# Autodesk Inventor assembly: J005189
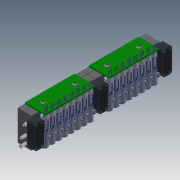
[picture p0: Inventor's stored thumbnail of the model, 180x180]
Saved by Autodesk Inventor 2020 (Build 240168000, 168)
## iProperties
RuleStatus: InUse
Created: 2015-04-18
Vendor: HHMI: JRC - ID&F
Document SubType Name: Assembly
Designer: JORDANJ
Part Number: J005189
Description: COMPONENT OF AN AUTOMATED LIQUID HANDLING MACHINE SPECIFICALLY DESIGNED FOR THE IN SITU RNA HYBRIDIZATION OF DROSOPHILA EMBRYOS
Project: P-171601
AfterDocSave0: file://Part Number Cleaner
DESIGN DEPARTMENT: HHMI: JRC - ID&F
LAB/DEPT: STERN (LAB)
REQUESTING SCIENTIST: STERN, DAVID
SPECIAL FINISH: NONE
SURFACE ROUGHNESS: N/A
ALTERED ITEM PART NUMBER: N/A
ALTERED ITEM VENDOR: N/A
ALTERED ITEM DESCRIPTION: N/A
Revision Number: 0
## Documents named in this file (4)
- C:\_WORKSPACE\DATA\PROJECTS\_PROJECTS BY LAB\STERN (LAB)\HYBRIDIZER\MCAD\MICROPLATE\24W CHEMICAL MANIFOLD ASSY.iam
- C:\_WORKSPACE\DATA\PROJECTS\_PROJECTS BY LAB\STERN (LAB)\HYBRIDIZER\MCAD\MICROPLATE\24W CHEMICAL MANIFOLD.iam
- C:\_WORKSPACE\DATA\PROJECTS\_PROJECTS BY LAB\STERN (LAB)\HYBRIDIZER\MCAD\MICROPLATE\24W CHEM MANIFOLD MOUNT.ipt
- C:\_WORKSPACE\DATA\PROJECTS\_PROJECTS BY LAB\STERN (LAB)\HYBRIDIZER\MCAD\MICROPLATE\24W CHEM MANIFOLD ORING.ipt
## Components (8 placed, 3 different names)
1. 24W CHEM MANIFOLD MOUNT:1 — Flush:6, Flush:7, Flush:8, Insert:3, Insert:4
2. 24W CHEMICAL MANIFOLD:1 [sub-assembly] — Mate:1, Flush:3, Flush:4, Flush:5, Insert:3, Insert:4, Mate:2, Mate:3, Mate:4, Flush:9, Flush:10, Flush:11
3. 24W CHEMICAL MANIFOLD:2 [sub-assembly] — Mate:1, Insert:1, Insert:2, Insert:5, Insert:6
4. 24W CHEM MANIFOLD MOUNT:2 — Insert:5, Insert:6
5. 24W CHEM MANIFOLD MOUNT:3 — Insert:1, Insert:2
6. 24W CHEM MANIFOLD ORING:1 — Mate:4, Flush:9
7. 24W CHEM MANIFOLD ORING:2 — Mate:2, Flush:11
8. 24W CHEM MANIFOLD ORING:3 — Mate:3, Flush:10
## Relationships (21: Flush 11, Insert 6, Mate 4)
- [Flush]: 24W CHEMICAL MANIFOLD:1 ↔ 24W CHEMICAL MANIFOLD:2
- [Flush]: 24W CHEMICAL MANIFOLD:1 ↔ 24W CHEMICAL MANIFOLD:2
- Mate:1: 24W CHEMICAL MANIFOLD:1 ↔ 24W CHEMICAL MANIFOLD:2
- Flush:3: 24W CHEMICAL MANIFOLD:1
- Flush:4: 24W CHEMICAL MANIFOLD:1
- Flush:5: 24W CHEMICAL MANIFOLD:1
- Flush:6: 24W CHEM MANIFOLD MOUNT:1
- Flush:7: 24W CHEM MANIFOLD MOUNT:1
- Flush:8: 24W CHEM MANIFOLD MOUNT:1
- Insert:1: 24W CHEMICAL MANIFOLD:2 ↔ 24W CHEM MANIFOLD MOUNT:3
- Insert:2: 24W CHEMICAL MANIFOLD:2 ↔ 24W CHEM MANIFOLD MOUNT:3
- Insert:3: 24W CHEM MANIFOLD MOUNT:1 ↔ 24W CHEMICAL MANIFOLD:1
- Insert:4: 24W CHEM MANIFOLD MOUNT:1 ↔ 24W CHEMICAL MANIFOLD:1
- Insert:5: 24W CHEMICAL MANIFOLD:2 ↔ 24W CHEM MANIFOLD MOUNT:2
- Insert:6: 24W CHEMICAL MANIFOLD:2 ↔ 24W CHEM MANIFOLD MOUNT:2
- Mate:2: 24W CHEMICAL MANIFOLD:1 ↔ 24W CHEM MANIFOLD ORING:2
- Mate:3: 24W CHEMICAL MANIFOLD:1 ↔ 24W CHEM MANIFOLD ORING:3
- Mate:4: 24W CHEMICAL MANIFOLD:1 ↔ 24W CHEM MANIFOLD ORING:1
- Flush:9: 24W CHEMICAL MANIFOLD:1 ↔ 24W CHEM MANIFOLD ORING:1
- Flush:10: 24W CHEMICAL MANIFOLD:1 ↔ 24W CHEM MANIFOLD ORING:3
- Flush:11: 24W CHEMICAL MANIFOLD:1 ↔ 24W CHEM MANIFOLD ORING:2
## Named parameters: d65_d43 = 0 mm
